# Autodesk Inventor assembly: Assembly_UR3GRIP
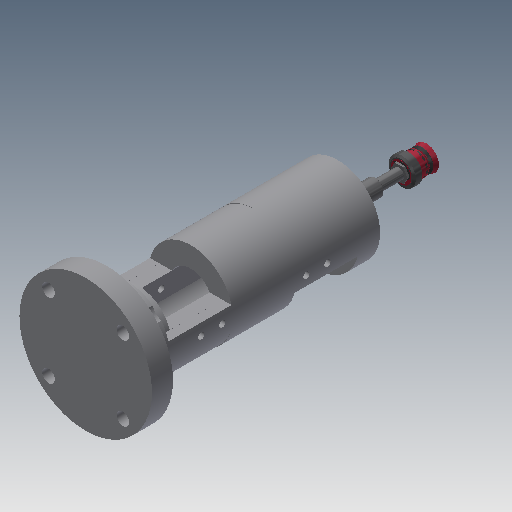
[picture p0: Inventor's stored thumbnail of the model, 512x512]
Saved by Autodesk Inventor 2019 (Build 230136000, 136)
## iProperties
Created: 2019-07-25
Part Number: Assembly_UR3GRIP
Document SubType Name: Assembly
Designer: romanp
Author: romanp
## Documents named in this file (6)
- C:\Users\romanp\Desktop\i4C_model\Pack_and_Go\Assembly_UR3GRIP.iam
- C:\Users\romanp\Desktop\i4C_model\Pack_and_Go\Part2_abbGripp.ipt
- C:\Users\romanp\Desktop\i4C_model\Pack_and_Go\Part3_abbGripp.ipt
- C:\Users\romanp\Desktop\i4C_model\Pack_and_Go\Part1_ur3Gripp.ipt
- C:\Users\romanp\Desktop\i4C_model\Pack_and_Go\ZP3-T10BSJ10-B5.iam
- C:\Users\romanp\Desktop\i4C_model\Pack_and_Go\ZPR20UNK10-06-A10.step_ZPR7011 Nut_10-32.ipt
## Components (6 placed, 5 different names)
1. Part2_abbGripp:1 — Insert:2, Insert:3
2. Part3_abbGripp:1 — Insert:2, Insert:7
3. Part1_ur3Gripp:1 — Insert:3
4. ZPR20UNK10-06-A10.step_ZPR7011 Nut_10-32:1 — Insert:4, Insert:5, Insert:6
5. ZP3-T10BSJ10-B5:1 [sub-assembly] — Insert:4, Insert:5
6. ZPR20UNK10-06-A10.step_ZPR7011 Nut_10-32:2 — Insert:6, Insert:7
## Relationships (6: Insert 6)
- Insert:2: Part2_abbGripp:1 ↔ Part3_abbGripp:1
- Insert:3: Part2_abbGripp:1 ↔ Part1_ur3Gripp:1
- Insert:4: ZPR20UNK10-06-A10.step_ZPR7011 Nut_10-32:1 ↔ ZP3-T10BSJ10-B5:1
- Insert:5: ZPR20UNK10-06-A10.step_ZPR7011 Nut_10-32:1 ↔ ZP3-T10BSJ10-B5:1
- Insert:6 (-0.24 mm): ZPR20UNK10-06-A10.step_ZPR7011 Nut_10-32:1 ↔ ZPR20UNK10-06-A10.step_ZPR7011 Nut_10-32:2
- Insert:7: Part3_abbGripp:1 ↔ ZPR20UNK10-06-A10.step_ZPR7011 Nut_10-32:2
